# Autodesk Inventor assembly: Wheel Assembly
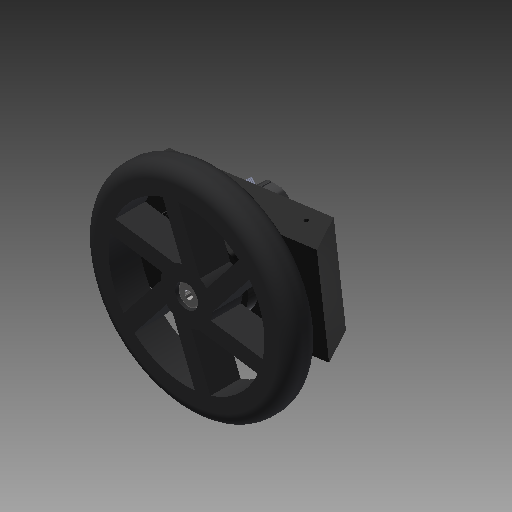
[picture p0: Inventor's stored thumbnail of the model, 512x512]
Saved by Autodesk Inventor 2017 (Build 210142000, 142)
## iProperties
Created: 2018-10-18
Part Number: Wheel Assembly
Document SubType Name: Assembly
Designer: Dell
Author: Dell
## Documents named in this file (7)
- C:\Users\Dell\Documents\GitHub\tr2\Wheel Assembly\Wheel Assembly, Right.iam
- C:\Users\Dell\Documents\GitHub\tr2\Wheel Assembly\Scooter Wheel.ipt
- C:\Users\Dell\Documents\GitHub\tr2\Wheel Assembly\WA01.ipt
- C:\Users\Dell\Documents\GitHub\tr2\Wheel Assembly\Wheel Assembly\Design Accelerator\Spur Gears1.iam
- C:\Users\Dell\Documents\GitHub\tr2\Base\37d-gearmotor-50-70-encoder.ipt
- C:\Users\Dell\Documents\GitHub\tr2\Wheel Assembly\22x8x8mm Bearing.ipt
- C:\Users\Dell\Documents\GitHub\tr2\Wheel Assembly\6mm Mounting Hub, thin.ipt
## Components (12 placed, 6 different names)
1. Scooter Wheel:1 — Mate:25, Mate:26, Mate:27, Mate:28, Mate:47, Rotation:1
2. WA01:1 — Mate:9, Mate:10, Mate:11, Mate:36, Mate:39, Mate:40, Mate:42, Mate:43, Mate:44, Mate:46
3. Spur Gears:1 [sub-assembly] — Mate:21, Mate:22, Mate:44, Mate:45, Mate:46, Mate:47, Rotation:1, Mate:48, Mate:49, Mate:50
4. 37d-gearmotor-50-70-encoder:1 — Mate:9, Mate:10, Mate:11, Mate:20, Mate:45
5. 22x8x8mm Bearing:1 — Mate:37, Mate:48
6. 22x8x8mm Bearing:2 — Mate:36, Mate:37, Mate:49
7. 6mm Mounting Hub, thin:1 — Mate:20, Mate:21, Mate:22
8. 22x8x8mm Bearing:3 — Mate:34, Mate:41
9. 22x8x8mm Bearing:4 — Mate:25, Mate:26
10. 22x8x8mm Bearing:5 — Mate:27, Mate:28, Mate:34, Mate:50
11. 22x8x8mm Bearing:6 — Mate:39, Mate:40, Mate:41
12. 22x8x8mm Bearing:7 — Mate:42, Mate:43
## Relationships (26: Mate 25, RelateRotation 1)
- Mate:9: WA01:1 ↔ 37d-gearmotor-50-70-encoder:1
- Mate:10: WA01:1 ↔ 37d-gearmotor-50-70-encoder:1
- Mate:11: WA01:1 ↔ 37d-gearmotor-50-70-encoder:1
- Mate:20: 37d-gearmotor-50-70-encoder:1 ↔ 6mm Mounting Hub, thin:1
- Mate:21: Spur Gears:1 ↔ 6mm Mounting Hub, thin:1
- Mate:22: Spur Gears:1 ↔ 6mm Mounting Hub, thin:1
- Mate:25: Scooter Wheel:1 ↔ 22x8x8mm Bearing:4
- Mate:26: Scooter Wheel:1 ↔ 22x8x8mm Bearing:4
- Mate:27: Scooter Wheel:1 ↔ 22x8x8mm Bearing:5
- Mate:28: Scooter Wheel:1 ↔ 22x8x8mm Bearing:5
- Mate:34: 22x8x8mm Bearing:3 ↔ 22x8x8mm Bearing:5
- Mate:36: WA01:1 ↔ 22x8x8mm Bearing:2
- Mate:37: 22x8x8mm Bearing:1 ↔ 22x8x8mm Bearing:2
- Mate:39: WA01:1 ↔ 22x8x8mm Bearing:6
- Mate:40: WA01:1 ↔ 22x8x8mm Bearing:6
- Mate:41: 22x8x8mm Bearing:3 ↔ 22x8x8mm Bearing:6
- Mate:42: WA01:1 ↔ 22x8x8mm Bearing:7
- Mate:43: WA01:1 ↔ 22x8x8mm Bearing:7
- Mate:44: WA01:1 ↔ Spur Gears:1
- Mate:45: Spur Gears:1 ↔ 37d-gearmotor-50-70-encoder:1
- Mate:46: WA01:1 ↔ Spur Gears:1
- Mate:47: Scooter Wheel:1 ↔ Spur Gears:1
- Rotation:1 [RelateRotation] (1 ul): Scooter Wheel:1 ↔ Spur Gears:1
- Mate:48: Spur Gears:1 ↔ 22x8x8mm Bearing:1
- Mate:49: Spur Gears:1 ↔ 22x8x8mm Bearing:2
- Mate:50: Spur Gears:1 ↔ 22x8x8mm Bearing:5
